# Autodesk Inventor assembly: Ensamblaje
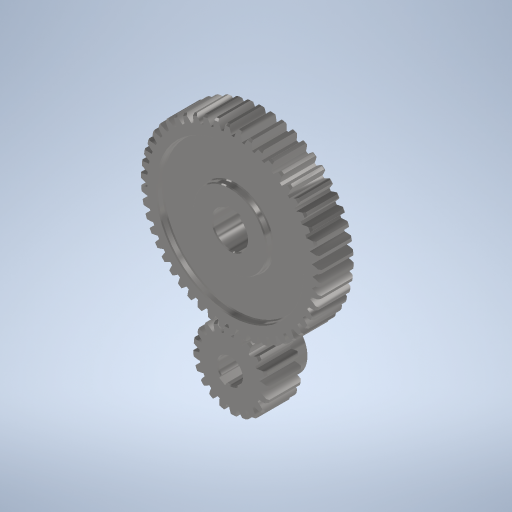
[picture p0: Inventor's stored thumbnail of the model, 512x512]
Saved by Autodesk Inventor 2024 (Build 280153000, 153)
## iProperties
Created: 2023-12-10
Part Number: Ensamblaje
Document SubType Name: Assembly
Designer: Jhon
Author: Jhon
## Documents named in this file (2)
- C:\Users\Jhon\Desktop\MSGA(B) Ground Spur Gears KHK\Ensamblaje.iam
- C:\Users\Jhon\Desktop\MSGA(B) Ground Spur Gears KHK\Engranajes rectos1.iam
## Components (1 placed, 1 different names)
1. Engranajes rectos:1 [sub-assembly] — Coincidencia:2, Coincidencia:3, Coincidencia:4, Nivelación:1
## Relationships (4: Mate 3, Flush 1)
- Coincidencia:2 [Mate]: Engranajes rectos:1
- Coincidencia:3 [Mate]: Engranajes rectos:1
- Coincidencia:4 [Mate]: Engranajes rectos:1
- Nivelación:1 [Flush]: Engranajes rectos:1
